# Autodesk Inventor assembly: 4_Camera
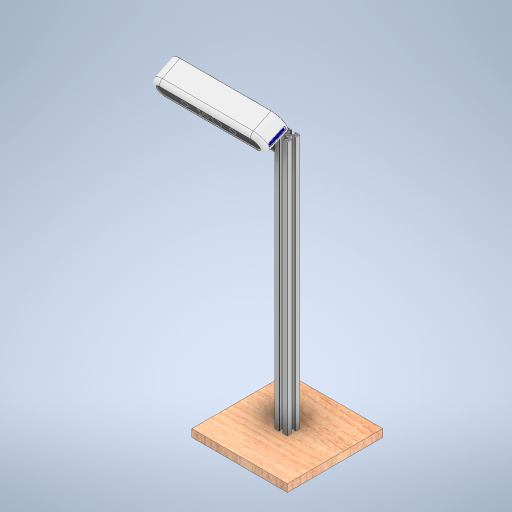
[picture p0: Inventor's stored thumbnail of the model, 512x512]
Saved by Autodesk Inventor 2024.2 (Build 282272000, 272)
## iProperties
Created: 2023-11-26
Part Number: 4_Camera
Document SubType Name: Assembly
Designer: 박동준
Author: 박동준
## Documents named in this file (8)
- C:\Users\박동준\OneDrive - 연세대학교 (Yonsei University)\바탕 화면\박동준\대학생할\로봇\Humanoid\7축 매니퓰레이터\하드웨어\rh_plus_7_axis_robot_arm_hardware\Assembly\4_Camera.iam
- C:\Users\박동준\OneDrive - 연세대학교 (Yonsei University)\바탕 화면\박동준\대학생할\로봇\Humanoid\7축 매니퓰레이터\하드웨어\rh_plus_7_axis_robot_arm_hardware\Part\Other Parts\Aluminum_Profile_2020_400mm.ipt
- C:\Users\박동준\OneDrive - 연세대학교 (Yonsei University)\바탕 화면\박동준\대학생할\로봇\Humanoid\7축 매니퓰레이터\하드웨어\rh_plus_7_axis_robot_arm_hardware\Part\Other Parts\Aluminum_Profile_2020_150mm.ipt
- C:\Users\박동준\OneDrive - 연세대학교 (Yonsei University)\바탕 화면\박동준\대학생할\로봇\Humanoid\7축 매니퓰레이터\하드웨어\rh_plus_7_axis_robot_arm_hardware\Part\Other Parts\Camera_base_plate.ipt
- C:\Users\박동준\OneDrive - 연세대학교 (Yonsei University)\바탕 화면\박동준\대학생할\로봇\Humanoid\7축 매니퓰레이터\하드웨어\rh_plus_7_axis_robot_arm_hardware\Part\Other Parts\Camera_mount.ipt
- C:\Users\박동준\OneDrive - 연세대학교 (Yonsei University)\바탕 화면\박동준\대학생할\로봇\Humanoid\7축 매니퓰레이터\하드웨어\rh_plus_7_axis_robot_arm_hardware\Part\Other Parts\Astra plus Camera.ipt
- C:\Users\박동준\OneDrive - 연세대학교 (Yonsei University)\바탕 화면\박동준\대학생할\로봇\Humanoid\7축 매니퓰레이터\하드웨어\rh_plus_7_axis_robot_arm_hardware\Part\Bolt, Bearing, Nut, Washer\M2.5x10 Round Bolt.ipt
- C:\Users\박동준\OneDrive - 연세대학교 (Yonsei University)\바탕 화면\박동준\대학생할\로봇\Humanoid\7축 매니퓰레이터\하드웨어\rh_plus_7_axis_robot_arm_hardware\Part\Bolt, Bearing, Nut, Washer\M4x10 Bolt.ipt
## Components (9 placed, 7 different names)
1. M2.5x10 Round Bolt:1 — Rigid:1
2. M2.5x10 Round Bolt:2 — Rigid:2
3. M4x10 Bolt:1 — Rigid:4
4. M4x10 Bolt:2 — Rigid:3
5. Astra plus Camera:1
6. Camera_mount:1 — Mate:13, Flush:1, Flush:2, Rigid:1, Rigid:2, Rigid:3, Rigid:4
7. Aluminum_Profile_2020_400mm:1 — Mate:1, Mate:2, Angle:2, Mate:3, Angle:3, Mate:4, Mate:5, Mate:8, Angle:4, Mate:9
8. Aluminum_Profile_2020_150mm:1 — Mate:3, Angle:3, Mate:4, Mate:5, Mate:13, Flush:1, Flush:2
9. Camera_base_plate:1 — Mate:8, Angle:4, Mate:9
## Relationships (22: Mate 11, Angle 5, WeldJoint 4, Flush 2)
- Mate:1: Aluminum_Profile_2020_400mm:1
- Mate:2: Aluminum_Profile_2020_400mm:1
- Angle:2 (0 deg): Aluminum_Profile_2020_400mm:1
- Mate:3: Aluminum_Profile_2020_400mm:1 ↔ Aluminum_Profile_2020_150mm:1
- Angle:3 (25 deg): Aluminum_Profile_2020_400mm:1 ↔ Aluminum_Profile_2020_150mm:1
- Mate:4: Aluminum_Profile_2020_400mm:1 ↔ Aluminum_Profile_2020_150mm:1
- Mate:5: Aluminum_Profile_2020_400mm:1 ↔ Aluminum_Profile_2020_150mm:1
- Mate:8: Aluminum_Profile_2020_400mm:1 ↔ Camera_base_plate:1
- Angle:4 (0 deg): Aluminum_Profile_2020_400mm:1 ↔ Camera_base_plate:1
- Mate:9: Aluminum_Profile_2020_400mm:1 ↔ Camera_base_plate:1
- [Angle] (0 deg): Camera_mount:1 ↔ Aluminum_Profile_2020_150mm:1
- [Angle] (0 deg): Camera_mount:1 ↔ Aluminum_Profile_2020_150mm:1
- [Mate]: Astra plus Camera:1 ↔ Camera_mount:1
- [Mate]: Astra plus Camera:1 ↔ Camera_mount:1
- [Mate]: Astra plus Camera:1 ↔ Camera_mount:1
- Mate:13: Camera_mount:1 ↔ Aluminum_Profile_2020_150mm:1
- Flush:1 (50 mm): Camera_mount:1 ↔ Aluminum_Profile_2020_150mm:1
- Flush:2 (5.8 mm): Camera_mount:1 ↔ Aluminum_Profile_2020_150mm:1
- Rigid:1 [WeldJoint]: M2.5x10 Round Bolt:1 ↔ Camera_mount:1
- Rigid:2 [WeldJoint]: M2.5x10 Round Bolt:2 ↔ Camera_mount:1
- Rigid:3 [WeldJoint]: M4x10 Bolt:2 ↔ Camera_mount:1
- Rigid:4 [WeldJoint]: M4x10 Bolt:1 ↔ Camera_mount:1
